# Autodesk Inventor assembly: MainAssembly
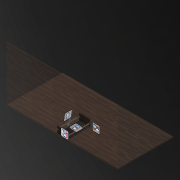
[picture p0: Inventor's stored thumbnail of the model, 180x180]
Saved by Autodesk Inventor 2019 (Build 230136000, 136)
## iProperties
Created: 2018-12-30
Part Number: MainAssembly
Document SubType Name: Assembly
Designer: JedrzejDankowski
Author: JedrzejDankowski
## Documents named in this file (10)
- C:\Users\MJ\Documents\AiFit-Inventor\MainAssembly.iam
- C:\Users\MJ\Documents\AiFit-Inventor\Arm.iam
- C:\Users\MJ\Documents\AiFit-Inventor\body.ipt
- C:\Users\MJ\Documents\groundpt.ipt
- C:\Users\MJ\Documents\AiFit-Inventor\motor.ipt
- C:\Users\MJ\Documents\AiFit-Inventor\pulley_dc.ipt
- C:\Users\MJ\Documents\AiFit-Inventor\pulley_small_pair.iam
- C:\Users\MJ\Documents\AiFit-Inventor\pad.ipt
- C:\Users\MJ\Documents\AiFit-Inventor\virsutinis.ipt
- C:\Users\MJ\Documents\AiFit-Inventor\pulley.ipt
## Components (12 placed, 9 different names)
1. body:1 — Flush:7, Mate:10, Flush:9, Rotational:1, Rotational:2, Mate:11, Mate:12, Mate:13, Mate:14, Mate:15
2. groundpt:1 — Flush:7, Mate:10, Flush:8
3. Arm:1 [sub-assembly] — Rotation:1, Flush:10, Rotational:1, Flush:12, Planar:1
4. pulley_small_pair:1 [sub-assembly]
5. pulley_dc:1 — Rotational:4
6. motor:1 — Mate:11, Flush:11, Mate:13, Rotational:4, Mate:14
7. virsutinis:1 — Rotational:7
8. pulley:1
9. pad:1 — Flush:12, Rotational:7, Planar:1
10. pulley_dc:2 — Rotational:3
11. motor:2 — Mate:12, Flush:11, Rotational:3, Mate:15
12. Arm:2 [sub-assembly] — Rotation:1, Flush:10, Rotational:2
## Relationships (21: RevoluteJoint 7, Flush 6, Mate 6, RelateRotation 1, PlanarJoint 1)
- Flush:7: body:1 ↔ groundpt:1
- Mate:10: body:1 ↔ groundpt:1
- Flush:8: groundpt:1
- Flush:9: body:1
- Rotation:1 [RelateRotation] (-1 ul): Arm:1 ↔ Arm:2
- Flush:10: Arm:1 ↔ Arm:2
- Rotational:1 [RevoluteJoint]: body:1 ↔ Arm:1
- Rotational:2 [RevoluteJoint]: body:1 ↔ Arm:2
- Mate:11: body:1 ↔ motor:1
- Mate:12: body:1 ↔ motor:2
- Flush:11: motor:1 ↔ motor:2
- Mate:13 (50 mm): body:1 ↔ motor:1
- Rotational:3 [RevoluteJoint] (-20 mm): pulley_dc:2 ↔ motor:2
- Rotational:4 [RevoluteJoint] (-20 mm): pulley_dc:1 ↔ motor:1
- Mate:14 (50 mm): body:1 ↔ motor:1
- Mate:15 (50 mm): body:1 ↔ motor:2
- [RevoluteJoint] (-25 mm): pulley_small_pair:1 ↔ virsutinis:1
- Flush:12: Arm:1 ↔ pad:1
- [RevoluteJoint] (-8 mm): virsutinis:1 ↔ pulley:1
- Rotational:7 [RevoluteJoint]: virsutinis:1 ↔ pad:1
- Planar:1: Arm:1 ↔ pad:1
